# Autodesk Inventor assembly: 6_right_arm_no error
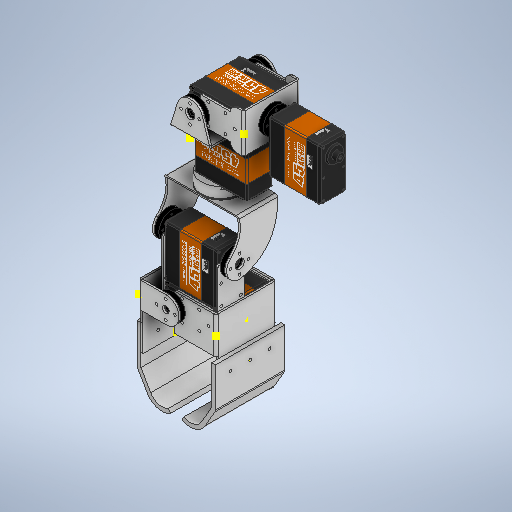
[picture p0: Inventor's stored thumbnail of the model, 512x512]
Saved by Autodesk Inventor 2025.2 (Build 292293000, 293)
## iProperties
Created: 2025-07-28
Part Number: 6_right_arm_no error
Document SubType Name: Assembly
Designer: LG
Author: LG
## Documents named in this file (15)
- C:\Users\LG\Desktop\RHp_Humanoid_ver1\Assembly\6_right_arm_no error.iam
- C:\Users\LG\Desktop\RHp_Humanoid_ver1\Part\HTD-45H, Horn\HTD-45H\HTD-45H.iam
- C:\Users\LG\Desktop\RHp_Humanoid_ver1\Part\HTD-45H, Horn\Horn\Top Horn.ipt
- C:\Users\LG\Desktop\RHp_Humanoid_ver1\Part\Frame\Arm\axis_19_top_frame.ipt
- C:\Users\LG\Desktop\RHp_Humanoid_ver1\Part\HTD-45H, Horn\Horn\Bottom Horn.ipt
- C:\Users\LG\Desktop\RHp_Humanoid_ver1\Part\Frame\Arm\axis_20_bottom_frame.ipt
- C:\Users\LG\Desktop\RHp_Humanoid_ver1\Part\Frame\Arm\axis_21_top_frame.ipt
- C:\Users\LG\Desktop\RHp_Humanoid_ver1\Part\Bolt, Bearing, Nut, Washer\2030 Teflon Sheet.ipt
- C:\Users\LG\Desktop\RHp_Humanoid_ver1\Part\Frame\Arm\axis_21_bottom_test_frame.ipt
- C:\Users\LG\Desktop\RHp_Humanoid_ver1\Part\Frame\Arm\axis_22_top_frame.ipt
- C:\Users\LG\Desktop\RHp_Humanoid_ver1\Part\Frame\Arm\axis_22_bottom_frame.ipt
- C:\Users\LG\Desktop\RHp_Humanoid_ver1\Part\Frame\Arm\axis_23_bottom_frame.ipt
- C:\Users\LG\Desktop\RHp_Humanoid_ver1\Part\Frame\Arm\axis_23_top_frame.ipt
- C:\Users\LG\Desktop\RHp_Humanoid_ver1\Part\Frame\Arm\HTD-45H_no bottom horn.ipt
- C:\Users\LG\Desktop\RHp_Humanoid_ver1\Part\Frame\Arm\gripper_frame.ipt
## Components (25 placed, 13 different names)
1. HTD-45H:1 [sub-assembly] — Mate:1, Mate:2, Mate:3, Rotational:1
2. Top Horn:1 — Rotational:1, Mate:6, Mate:14, Mate:15
3. axis_19_top_frame:1 — Mate:6, Mate:7, Mate:8, Mate:9, Mate:14, Mate:15
4. Bottom Horn:1 — Mate:10, Mate:11, Flush:1
5. HTD-45H:2 [sub-assembly] — Mate:7, Mate:8, Mate:9, Rotational:2, Mate:10, Mate:11, Flush:1
6. Top Horn:2 — Rotational:2, Flush:2, Mate:12, Mate:13
7. axis_20_bottom_frame:1 — Flush:2, Mate:12, Mate:13, Mate:46, Flush:12, Flush:13
8. HTD-45H:6 — Mate:46, Flush:12, Flush:13, Rotational:6, Mate:47, Flush:14, Mate:48
9. Top Horn:3 — Mate:22, Flush:6, Mate:23, Rotational:6
10. axis_21_top_frame:1 — Mate:19, Mate:20, Mate:21, Mate:47, Flush:14, Mate:48
11. 2030 Teflon Sheet:1 — Mate:19, Mate:20, Mate:21, Mate:24, Mate:25
12. 2030 Teflon Sheet:2 — Mate:24, Mate:25, Mate:26
13. axis_21_bottom_test_frame:1 — Mate:22, Flush:6, Mate:23, Mate:26, Mate:29, Mate:30, Mate:31
14. Bottom Horn:2 — Mate:27, Flush:7, Mate:28
15. HTD-45H:4 [sub-assembly] — Mate:27, Flush:7, Mate:28, Rotational:4, Mate:35, Flush:8, Flush:9, Mate:37, Mate:38
16. Top Horn:4 — Rotational:4, Mate:29, Mate:30, Mate:31
17. Bottom Horn:3 — Mate:32, Mate:33, Mate:34
18. HTD-45H:5 [sub-assembly] — Rotational:5, Mate:32, Mate:33, Mate:34, Mate:35, Flush:8, Flush:9, Mate:36, Mate:40, Flush:10
19. Top Horn:5 — Rotational:5, Mate:41, Mate:42, Mate:43
20. axis_22_top_frame:1 — Mate:36, Mate:37, Mate:38, Mate:39, Mate:45
21. axis_22_bottom_frame:1 — Mate:39, Mate:40, Flush:10, Mate:44, Flush:11
22. axis_23_bottom_frame:1 — Mate:41, Mate:42, Mate:43, Rigid:1
23. axis_23_top_frame:1 — Mate:44, Flush:11, Mate:45, Cylindrical:1
24. gripper_frame:1 — Rigid:1
25. gripper_frame:2 — Cylindrical:1
## Relationships (61: Mate 43, Flush 11, RevoluteJoint 5, WeldJoint 1, CylindricalJoint 1)
- Mate:1: HTD-45H:1
- Mate:2: HTD-45H:1
- Mate:3: HTD-45H:1
- Rotational:1 [RevoluteJoint]: HTD-45H:1 ↔ Top Horn:1
- Mate:6: Top Horn:1 ↔ axis_19_top_frame:1
- Mate:7: axis_19_top_frame:1 ↔ HTD-45H:2
- Mate:8 (2.5 mm): axis_19_top_frame:1 ↔ HTD-45H:2
- Mate:9: axis_19_top_frame:1 ↔ HTD-45H:2
- Rotational:2 [RevoluteJoint]: HTD-45H:2 ↔ Top Horn:2
- Mate:10: Bottom Horn:1 ↔ HTD-45H:2
- Mate:11: Bottom Horn:1 ↔ HTD-45H:2
- Flush:1: Bottom Horn:1 ↔ HTD-45H:2
- Flush:2 (14.5 mm): Top Horn:2 ↔ axis_20_bottom_frame:1
- Mate:12: Top Horn:2 ↔ axis_20_bottom_frame:1
- Mate:13: Top Horn:2 ↔ axis_20_bottom_frame:1
- Mate:14: Top Horn:1 ↔ axis_19_top_frame:1
- Mate:15: Top Horn:1 ↔ axis_19_top_frame:1
- Mate:19: axis_21_top_frame:1 ↔ 2030 Teflon Sheet:1
- Mate:20: axis_21_top_frame:1 ↔ 2030 Teflon Sheet:1
- Mate:21: axis_21_top_frame:1 ↔ 2030 Teflon Sheet:1
- Mate:22: Top Horn:3 ↔ axis_21_bottom_test_frame:1
- Flush:6: Top Horn:3 ↔ axis_21_bottom_test_frame:1
- Mate:23: Top Horn:3 ↔ axis_21_bottom_test_frame:1
- Mate:24: 2030 Teflon Sheet:1 ↔ 2030 Teflon Sheet:2
- Mate:25: 2030 Teflon Sheet:1 ↔ 2030 Teflon Sheet:2
- Mate:26: 2030 Teflon Sheet:2 ↔ axis_21_bottom_test_frame:1
- Mate:27: Bottom Horn:2 ↔ HTD-45H:4
- Flush:7: Bottom Horn:2 ↔ HTD-45H:4
- Mate:28: Bottom Horn:2 ↔ HTD-45H:4
- Rotational:4 [RevoluteJoint]: HTD-45H:4 ↔ Top Horn:4
- Mate:29 (30.43 mm): axis_21_bottom_test_frame:1 ↔ Top Horn:4
- Mate:30 (-14 mm): axis_21_bottom_test_frame:1 ↔ Top Horn:4
- Mate:31: axis_21_bottom_test_frame:1 ↔ Top Horn:4
- Rotational:5 [RevoluteJoint]: HTD-45H:5 ↔ Top Horn:5
- Mate:32: Bottom Horn:3 ↔ HTD-45H:5
- Mate:33: Bottom Horn:3 ↔ HTD-45H:5
- Mate:34: Bottom Horn:3 ↔ HTD-45H:5
- Mate:35: HTD-45H:4 ↔ HTD-45H:5
- Flush:8: HTD-45H:4 ↔ HTD-45H:5
- Flush:9: HTD-45H:4 ↔ HTD-45H:5
- Mate:36 (5 mm): HTD-45H:5 ↔ axis_22_top_frame:1
- Mate:37: HTD-45H:4 ↔ axis_22_top_frame:1
- Mate:38: HTD-45H:4 ↔ axis_22_top_frame:1
- Mate:39: axis_22_top_frame:1 ↔ axis_22_bottom_frame:1
- Mate:40: HTD-45H:5 ↔ axis_22_bottom_frame:1
- Flush:10: HTD-45H:5 ↔ axis_22_bottom_frame:1
- Mate:41: Top Horn:5 ↔ axis_23_bottom_frame:1
- Mate:42: Top Horn:5 ↔ axis_23_bottom_frame:1
- Mate:43 (19.43 mm): Top Horn:5 ↔ axis_23_bottom_frame:1
- Mate:44: axis_22_bottom_frame:1 ↔ axis_23_top_frame:1
- Flush:11: axis_22_bottom_frame:1 ↔ axis_23_top_frame:1
- Mate:45: axis_22_top_frame:1 ↔ axis_23_top_frame:1
- Mate:46: axis_20_bottom_frame:1 ↔ HTD-45H:6
- Flush:12: axis_20_bottom_frame:1 ↔ HTD-45H:6
- Flush:13: axis_20_bottom_frame:1 ↔ HTD-45H:6
- Rotational:6 [RevoluteJoint]: HTD-45H:6 ↔ Top Horn:3
- Mate:47: HTD-45H:6 ↔ axis_21_top_frame:1
- Flush:14: HTD-45H:6 ↔ axis_21_top_frame:1
- Mate:48: HTD-45H:6 ↔ axis_21_top_frame:1
- Rigid:1 [WeldJoint]: axis_23_bottom_frame:1 ↔ gripper_frame:1
- Cylindrical:1: axis_23_top_frame:1 ↔ gripper_frame:2
